# Autodesk Inventor assembly: DWG01
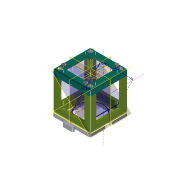
[picture p0: Inventor's stored thumbnail of the model, 180x180]
Saved by Autodesk Inventor 2022 (Build 260153000, 153)
## iProperties
Company: UC2
Created: 2018-06-11
Part Number: DWG01
Material: Generisch
Document SubType Name: Assembly
Designer: marsikova
Mass: 28.3962 g
Surface Area: 161.576 cm^2
Volume: 24.38 cm^3
Density: 1.16473 g/cm^3
Engineer: marsikova
Author: marsikova
Title: Assembly_Cube_empty_1x1_withBase_v3
Subject: Assembly_Cube_empty_1x1_withBase_v3
## Documents named in this file (7)
- C:\Users\PrakashLab\Documents\UC2-INVENTOR-Git\uc2_v3\Assembly_Cube_empty_1x1_withBase_v3.iam
- C:\Users\PrakashLab\Documents\UC2-INVENTOR-Git\uc2_v3\10_Cube_1x1_v3.ipt
- C:\Users\PrakashLab\Documents\UC2-INVENTOR-Git\uc2_v3\10_Lid_1x1_v3.ipt
- C:\Users\PrakashLab\Documents\UC2-INVENTOR-Git\uc2_v3\10_Base_puzzle_v3.ipt
- C:\Users\PrakashLab\Documents\UC2-INVENTOR-Git\uc2_v3\00_BallMagnets_5mm.ipt
- C:\Users\PrakashLab\Documents\Inventor\Content Center Files\R2022\en-US\ISO 4026\ISO 4026 - M5 x 8 - ISO.ipt
- C:\Users\PrakashLab\Documents\UC2-INVENTOR-Git\uc2_v3\DIN 912 - M3 x 0.5 x 12 x 10.75.ipt
## Components (18 placed, 6 different names)
1. 10_Cube_1x1_v3:1 — Mate:3, Mate:2, Angle:3, Mate:14, Angle:4, Mate:15, Symmetrie:1, Mate:19, Mate:20, Mate:21, Flush:8, Mate:25, Mate:26, Mate:27, Mate:28, Flush:15
2. 10_Lid_1x1_v3:1 — Mate:3, Mate:2, Flush:3, Flush:4, Flush:5, Insert:20, Insert:21, Insert:22, Insert:23, Angle:3, Symmetrie:1, Mate:22, Mate:23, Mate:24, Flush:11
3. DIN 912 - replaced by DIN EN ISO 4762 M3 x 12:5 — Insert:21
4. DIN 912 - replaced by DIN EN ISO 4762 M3 x 12:6 — Insert:23
5. DIN 912 - replaced by DIN EN ISO 4762 M3 x 12:7 — Insert:20
6. DIN 912 - replaced by DIN EN ISO 4762 M3 x 12:8 — Insert:22
7. 10_Base_puzzle_v3:1 — Mate:14, Angle:4, Mate:15, Mate:16, Mate:17, Tangent:1, Mate:18, Tangent:2
8. 00_BallMagnets_5mm:1 — Mate:16, Mate:17, Tangent:1, Mate:18, Tangent:2
9. ISO 4026 M5 x 8:1 — Mate:21, Flush:7
10. ISO 4026 M5 x 8:2 — Mate:22, Flush:9, Flush:10, Flush:11
11. ISO 4026 M5 x 8:3 — Mate:23, Flush:9
12. ISO 4026 M5 x 8:4 — Mate:20, Flush:6
13. ISO 4026 M5 x 8:5 — Mate:19, Flush:6, Flush:7, Flush:8
14. ISO 4026 M5 x 8:6 — Mate:24, Flush:10
15. DIN 912 - replaced by DIN EN ISO 4762 M3 x 12:1 — Mate:25, Flush:12, Flush:13, Flush:14, Flush:15
16. DIN 912 - replaced by DIN EN ISO 4762 M3 x 12:2 — Mate:28, Flush:13
17. DIN 912 - replaced by DIN EN ISO 4762 M3 x 12:3 — Mate:27, Flush:14
18. DIN 912 - replaced by DIN EN ISO 4762 M3 x 12:4 — Mate:26, Flush:12
## Relationships (39: Mate 17, Flush 13, Insert 4, Angle 2, Tangent 2, Symmetry 1)
- Mate:3: 10_Cube_1x1_v3:1 ↔ 10_Lid_1x1_v3:1
- Mate:2: 10_Cube_1x1_v3:1 ↔ 10_Lid_1x1_v3:1
- Flush:3: 10_Lid_1x1_v3:1
- Flush:4: 10_Lid_1x1_v3:1
- Flush:5: 10_Lid_1x1_v3:1
- Insert:20: 10_Lid_1x1_v3:1 ↔ DIN 912 - replaced by DIN EN ISO 4762 M3 x 12:7
- Insert:21: 10_Lid_1x1_v3:1 ↔ DIN 912 - replaced by DIN EN ISO 4762 M3 x 12:5
- Insert:22: 10_Lid_1x1_v3:1 ↔ DIN 912 - replaced by DIN EN ISO 4762 M3 x 12:8
- Insert:23: 10_Lid_1x1_v3:1 ↔ DIN 912 - replaced by DIN EN ISO 4762 M3 x 12:6
- Angle:3 (0 deg): 10_Cube_1x1_v3:1 ↔ 10_Lid_1x1_v3:1
- Mate:14: 10_Cube_1x1_v3:1 ↔ 10_Base_puzzle_v3:1
- Angle:4 (0 deg): 10_Cube_1x1_v3:1 ↔ 10_Base_puzzle_v3:1
- Mate:15: 10_Cube_1x1_v3:1 ↔ 10_Base_puzzle_v3:1
- Symmetrie:1: 10_Cube_1x1_v3:1 ↔ 10_Lid_1x1_v3:1
- Mate:16: 10_Base_puzzle_v3:1 ↔ 00_BallMagnets_5mm:1
- Mate:17: 10_Base_puzzle_v3:1 ↔ 00_BallMagnets_5mm:1
- Tangent:1: 10_Base_puzzle_v3:1 ↔ 00_BallMagnets_5mm:1
- Mate:18: 10_Base_puzzle_v3:1 ↔ 00_BallMagnets_5mm:1
- Tangent:2: 10_Base_puzzle_v3:1 ↔ 00_BallMagnets_5mm:1
- Mate:19: 10_Cube_1x1_v3:1 ↔ ISO 4026 M5 x 8:5
- Mate:20: 10_Cube_1x1_v3:1 ↔ ISO 4026 M5 x 8:4
- Mate:21: 10_Cube_1x1_v3:1 ↔ ISO 4026 M5 x 8:1
- Flush:6: ISO 4026 M5 x 8:4 ↔ ISO 4026 M5 x 8:5
- Flush:7: ISO 4026 M5 x 8:1 ↔ ISO 4026 M5 x 8:5
- Flush:8 (-2 mm): 10_Cube_1x1_v3:1 ↔ ISO 4026 M5 x 8:5
- Mate:22: 10_Lid_1x1_v3:1 ↔ ISO 4026 M5 x 8:2
- Mate:23: 10_Lid_1x1_v3:1 ↔ ISO 4026 M5 x 8:3
- Mate:24: 10_Lid_1x1_v3:1 ↔ ISO 4026 M5 x 8:6
- Flush:9: ISO 4026 M5 x 8:2 ↔ ISO 4026 M5 x 8:3
- Flush:10: ISO 4026 M5 x 8:2 ↔ ISO 4026 M5 x 8:6
- Flush:11 (-2 mm): 10_Lid_1x1_v3:1 ↔ ISO 4026 M5 x 8:2
- Mate:25: 10_Cube_1x1_v3:1 ↔ DIN 912 - replaced by DIN EN ISO 4762 M3 x 12:1
- Mate:26: 10_Cube_1x1_v3:1 ↔ DIN 912 - replaced by DIN EN ISO 4762 M3 x 12:4
- Mate:27: 10_Cube_1x1_v3:1 ↔ DIN 912 - replaced by DIN EN ISO 4762 M3 x 12:3
- Mate:28: 10_Cube_1x1_v3:1 ↔ DIN 912 - replaced by DIN EN ISO 4762 M3 x 12:2
- Flush:12: DIN 912 - replaced by DIN EN ISO 4762 M3 x 12:1 ↔ DIN 912 - replaced by DIN EN ISO 4762 M3 x 12:4
- Flush:13: DIN 912 - replaced by DIN EN ISO 4762 M3 x 12:1 ↔ DIN 912 - replaced by DIN EN ISO 4762 M3 x 12:2
- Flush:14: DIN 912 - replaced by DIN EN ISO 4762 M3 x 12:1 ↔ DIN 912 - replaced by DIN EN ISO 4762 M3 x 12:3
- Flush:15: 10_Cube_1x1_v3:1 ↔ DIN 912 - replaced by DIN EN ISO 4762 M3 x 12:1
